# Autodesk Inventor assembly: Rail_AssemblyV2_0
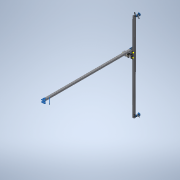
[picture p0: Inventor's stored thumbnail of the model, 180x180]
Saved by Autodesk Inventor 2021 (Build 250183000, 183)
## iProperties
Created: 2021-01-25
Part Number: Rail_AssemblyV2_0
Document SubType Name: Assembly
Designer: Jorian Brusind
Mass: 3786.54 g
Surface Area: 19508.5 cm^2
Volume: 2323.9 cm^3
Density: 1.62939 g/cm^3
Author: Jorian Brusind
## Documents named in this file (24)
- C:\Users\Jorian Brusind\Documents\GitHub\PersonalProjects\HyperRail\Inventor Files\Rail_AssemblyV2_0.iam
- C:\Users\Jorian Brusind\Documents\GitHub\PersonalProjects\Inventor Projects\Useful models\NEMA_Steppers\NEMA23\23HS8430B.ipt
- C:\Users\Jorian Brusind\Documents\GitHub\PersonalProjects\HyperRail\Inventor Files\NEMA23_StepperonlineMount.ipt
- C:\Users\Jorian Brusind\Documents\GitHub\PersonalProjects\Inventor Projects\Useful models\8020_Sets\IPT_20_Series\IPT_20_Series\20-2040_200mm.ipt
- C:\Users\Jorian Brusind\Documents\GitHub\PersonalProjects\HyperRail\Inventor Files\2804S_NEMA2115_1Gearbox.ipt
- C:\Users\Jorian Brusind\Documents\GitHub\PersonalProjects\Inventor Projects\Useful models\8020_Sets\IPT_40_Series\Extra_40_Series\90deg_4040.ipt
- C:\Users\Jorian Brusind\Documents\GitHub\PersonalProjects\HyperRail\Inventor Files\SmallBelt_LargePulley.ipt
- C:\Users\Jorian Brusind\Documents\GitHub\PersonalProjects\HyperRail\Inventor Files\Small_belt_5mm_1mm.ipt
- C:\Users\Jorian Brusind\Documents\GitHub\PersonalProjects\HyperRail\PCB Files\Integrated Stepper Motor Driver\ExportSTEP\Main.iam
- C:\Users\Jorian Brusind\Documents\GitHub\PersonalProjects\HyperRail\Inventor Files\NEMA23_Shroud.ipt
- C:\Users\Jorian Brusind\Documents\GitHub\PersonalProjects\Inventor Projects\Useful models\8020_Sets\IPT_20_Series\IPT_20_Series\20-4040_2m.ipt
- C:\Users\Jorian Brusind\Documents\GitHub\PersonalProjects\HyperRail\Inventor Files\98952A059_ALUM MALE-FEM THRDED HEX STANDOFF.ipt
- C:\Users\Jorian Brusind\Documents\GitHub\PersonalProjects\HyperRail\Inventor Files\95783A039_NYLON 6-6 MALE-FEM THRDED HEX STANDOFF.ipt
- C:\Users\Jorian Brusind\Documents\GitHub\PersonalProjects\HyperRail\Inventor Files\Integrated_Stepper_NEMA23_Mount.ipt
- C:\Users\Jorian Brusind\Documents\GitHub\PersonalProjects\HyperRail\Inventor Files\Foot_Spacer.ipt
- C:\Users\Jorian Brusind\Documents\GitHub\PersonalProjects\Inventor Projects\Useful models\Metric bolt\Bolt M5 50mm.ipt
- C:\Users\Jorian Brusind\Documents\GitHub\PersonalProjects\Inventor Projects\Useful models\Metric nuts\Nut M5.ipt
- C:\Users\Jorian Brusind\Documents\GitHub\PersonalProjects\HyperRail\Inventor Files\Bottom_Foot.ipt
- C:\Users\Jorian Brusind\Documents\GitHub\PersonalProjects\HyperRail\Inventor Files\120deg_Tslot_Gusset.ipt
- C:\Users\Jorian Brusind\Documents\GitHub\PersonalProjects\HyperRail\Inventor Files\90deg_4040Bracket.ipt
- C:\Users\Jorian Brusind\Documents\GitHub\PersonalProjects\HyperRail\Inventor Files\X_Carriage_V2_0.iam
- C:\Users\Jorian Brusind\Documents\GitHub\PersonalProjects\HyperRail\Inventor Files\11mm_BearingWheel.ipt
- C:\Users\Jorian Brusind\Documents\GitHub\PersonalProjects\HyperRail\Inventor Files\X_CarriageR_V2_0.iam
- C:\Users\Jorian Brusind\Documents\GitHub\PersonalProjects\HyperRail\Inventor Files\4mm_Roller_Spacer.ipt
## Components (40 placed, 23 different names)
1. 23HS8430B:1 — Mate:127, Angle:3, Mate:158, Mate:177, Mate:179, Mate:180, Mate:181, Mate:182, Mate:183, Mate:184, Mate:185, Mate:196, Mate:264, Mate:265
2. NEMA23_StepperonlineMount:1 — Angle:2, Mate:98, Mate:128, Mate:149, Mate:155, Flush:82, Mate:254, Mate:255, Mate:257, Mate:258, Mate:259, Mate:261, Mate:262
3. 20-2040_200mm:1 — Flush:34, Mate:83, Flush:35, Flush:36, Mate:85, Flush:56, Flush:63, Mate:151, Flush:82, Mate:252, Mate:253, Flush:83, Flush:84, Mate:256, Flush:85
4. 2804S_NEMA2115_1Gearbox:1 — Angle:2, Mate:98, Mate:109, Mate:127, Mate:128, Angle:3, Mate:158, Mate:204, Flush:66, Flush:86
5. 90deg_4040:1 — Flush:34, Mate:83, Flush:35, Mate:150
6. 90deg_4040:2 — Flush:36, Mate:85, Mate:149, Mate:152
7. SmallBelt_LargePulley:1 — Mate:204, Flush:66
8. Small_belt_5mm_1mm:1 — Mate:109, Flush:42, Mate:111, Flush:64
9. Small_belt_5mm_1mm:2 — Flush:42, Mate:111, Mate:154, Flush:64, Mate:205
10. Main:1 [sub-assembly] — Mate:199, Mate:267, Mate:268
11. 20-4040_2m:1 — Mate:139, Flush:56, Mate:154, Mate:205, Mate:243, Flush:76, Flush:77, Mate:248, Flush:79, Flush:80, Mate:252
12. 20-4040_2m:2 — Mate:150, Flush:63, Mate:151, Mate:152, Mate:155, Mate:230, Flush:69, Flush:70, Mate:231, Flush:71, Flush:72, Mate:232, Flush:73, Mate:233, Mate:234, Flush:74
13. NEMA23_Shroud:1 — Mate:264, Mate:265, Flush:86
14. 98952A059_ALUM MALE-FEM THRDED HEX STANDOFF:1 — Mate:180, Mate:181, Mate:186, Mate:191
15. 98952A059_ALUM MALE-FEM THRDED HEX STANDOFF:2 — Mate:184, Mate:185, Mate:189, Mate:192
16. 98952A059_ALUM MALE-FEM THRDED HEX STANDOFF:3 — Mate:177, Mate:179, Mate:187, Mate:190
17. 98952A059_ALUM MALE-FEM THRDED HEX STANDOFF:4 — Mate:182, Mate:183, Mate:188, Mate:193
18. 95783A039_NYLON 6-6 MALE-FEM THRDED HEX STANDOFF:1 — Mate:188, Mate:193, Angle:4
19. 95783A039_NYLON 6-6 MALE-FEM THRDED HEX STANDOFF:2 — Mate:186, Mate:191
20. 95783A039_NYLON 6-6 MALE-FEM THRDED HEX STANDOFF:3 — Mate:187, Mate:190, Mate:200
21. 95783A039_NYLON 6-6 MALE-FEM THRDED HEX STANDOFF:4 — Mate:189, Mate:192
22. Integrated_Stepper_NEMA23_Mount:1 — Mate:196, Mate:199, Mate:200, Angle:4, Mate:267, Mate:268
23. Bolt M5 50mm:1 — Mate:224, Mate:245, Mate:246, Mate:247, Mate:269
24. Nut M5:1 — Mate:226, Mate:247
25. Nut M5:2 — Mate:244, Flush:78, Mate:246
26. Bottom_Foot:1 — Mate:224, Mate:226, Mate:245, Flush:81
27. 120deg_Tslot_Gusset:1 — Mate:230, Flush:69, Flush:70
28. 120deg_Tslot_Gusset:2 — Mate:231, Flush:71, Flush:72
29. 90deg_4040Bracket:1 — Mate:232, Flush:73, Mate:233, Flush:75
30. 90deg_4040Bracket:2 — Mate:234, Flush:74, Flush:75
31. Foot_Spacer:1 — Mate:243, Flush:76, Flush:77, Mate:244, Flush:78, Mate:269
32. Foot_Spacer:2 — Mate:248, Flush:79, Flush:80, Mate:250
33. Bottom_Foot:2 — Mate:249, Mate:251, Flush:81
34. Bolt M5 50mm:2 — Mate:249, Mate:250, Mate:251
35. X_Carriage_V2_0:1 [sub-assembly] — Mate:253, Flush:83, Flush:84
36. 11mm_BearingWheel:1 — Mate:254, Mate:255, Mate:260
37. X_CarriageR_V2_0:1 [sub-assembly] — Mate:256, Flush:85, Mate:257
38. 11mm_BearingWheel:2 — Mate:258, Mate:259, Mate:263
39. 4mm_Roller_Spacer:1 — Mate:260, Mate:261
40. 4mm_Roller_Spacer:2 — Mate:262, Mate:263
## Relationships (98: Mate 69, Flush 26, Angle 3)
- Angle:2 (0 deg): NEMA23_StepperonlineMount:1 ↔ 2804S_NEMA2115_1Gearbox:1
- Flush:34: 20-2040_200mm:1 ↔ 90deg_4040:1
- Mate:83: 20-2040_200mm:1 ↔ 90deg_4040:1
- Flush:35: 20-2040_200mm:1 ↔ 90deg_4040:1
- Flush:36: 20-2040_200mm:1 ↔ 90deg_4040:2
- Mate:85: 20-2040_200mm:1 ↔ 90deg_4040:2
- Mate:98: NEMA23_StepperonlineMount:1 ↔ 2804S_NEMA2115_1Gearbox:1
- Mate:109 (10 mm): 2804S_NEMA2115_1Gearbox:1 ↔ Small_belt_5mm_1mm:1
- Flush:42: Small_belt_5mm_1mm:1 ↔ Small_belt_5mm_1mm:2
- Mate:111 (20 mm): Small_belt_5mm_1mm:1 ↔ Small_belt_5mm_1mm:2
- Mate:127: 23HS8430B:1 ↔ 2804S_NEMA2115_1Gearbox:1
- Mate:128: NEMA23_StepperonlineMount:1 ↔ 2804S_NEMA2115_1Gearbox:1
- Mate:139: 20-4040_2m:1
- Flush:56: 20-2040_200mm:1 ↔ 20-4040_2m:1
- Mate:149 (30 mm): NEMA23_StepperonlineMount:1 ↔ 90deg_4040:2
- Mate:150: 90deg_4040:1 ↔ 20-4040_2m:2
- Flush:63: 20-2040_200mm:1 ↔ 20-4040_2m:2
- Mate:151: 20-2040_200mm:1 ↔ 20-4040_2m:2
- Mate:152: 90deg_4040:2 ↔ 20-4040_2m:2
- Mate:154 (-10 mm): Small_belt_5mm_1mm:2 ↔ 20-4040_2m:1
- Flush:64: Small_belt_5mm_1mm:1 ↔ Small_belt_5mm_1mm:2
- Mate:155: NEMA23_StepperonlineMount:1 ↔ 20-4040_2m:2
- Angle:3 (0 deg): 23HS8430B:1 ↔ 2804S_NEMA2115_1Gearbox:1
- Mate:158: 23HS8430B:1 ↔ 2804S_NEMA2115_1Gearbox:1
- Mate:177: 23HS8430B:1 ↔ 98952A059_ALUM MALE-FEM THRDED HEX STANDOFF:3
- Mate:179: 23HS8430B:1 ↔ 98952A059_ALUM MALE-FEM THRDED HEX STANDOFF:3
- Mate:180: 23HS8430B:1 ↔ 98952A059_ALUM MALE-FEM THRDED HEX STANDOFF:1
- Mate:181: 23HS8430B:1 ↔ 98952A059_ALUM MALE-FEM THRDED HEX STANDOFF:1
- Mate:182: 23HS8430B:1 ↔ 98952A059_ALUM MALE-FEM THRDED HEX STANDOFF:4
- Mate:183: 23HS8430B:1 ↔ 98952A059_ALUM MALE-FEM THRDED HEX STANDOFF:4
- Mate:184: 23HS8430B:1 ↔ 98952A059_ALUM MALE-FEM THRDED HEX STANDOFF:2
- Mate:185: 23HS8430B:1 ↔ 98952A059_ALUM MALE-FEM THRDED HEX STANDOFF:2
- Mate:186: 98952A059_ALUM MALE-FEM THRDED HEX STANDOFF:1 ↔ 95783A039_NYLON 6-6 MALE-FEM THRDED HEX STANDOFF:2
- Mate:187: 98952A059_ALUM MALE-FEM THRDED HEX STANDOFF:3 ↔ 95783A039_NYLON 6-6 MALE-FEM THRDED HEX STANDOFF:3
- Mate:188: 98952A059_ALUM MALE-FEM THRDED HEX STANDOFF:4 ↔ 95783A039_NYLON 6-6 MALE-FEM THRDED HEX STANDOFF:1
- Mate:189: 98952A059_ALUM MALE-FEM THRDED HEX STANDOFF:2 ↔ 95783A039_NYLON 6-6 MALE-FEM THRDED HEX STANDOFF:4
- Mate:190: 98952A059_ALUM MALE-FEM THRDED HEX STANDOFF:3 ↔ 95783A039_NYLON 6-6 MALE-FEM THRDED HEX STANDOFF:3
- Mate:191: 98952A059_ALUM MALE-FEM THRDED HEX STANDOFF:1 ↔ 95783A039_NYLON 6-6 MALE-FEM THRDED HEX STANDOFF:2
- Mate:192: 98952A059_ALUM MALE-FEM THRDED HEX STANDOFF:2 ↔ 95783A039_NYLON 6-6 MALE-FEM THRDED HEX STANDOFF:4
- Mate:193: 98952A059_ALUM MALE-FEM THRDED HEX STANDOFF:4 ↔ 95783A039_NYLON 6-6 MALE-FEM THRDED HEX STANDOFF:1
- Mate:196 (2 mm): 23HS8430B:1 ↔ Integrated_Stepper_NEMA23_Mount:1
- Mate:199 (1 mm): Main:1 ↔ Integrated_Stepper_NEMA23_Mount:1
- Mate:200: 95783A039_NYLON 6-6 MALE-FEM THRDED HEX STANDOFF:3 ↔ Integrated_Stepper_NEMA23_Mount:1
- Angle:4 (0 deg): 95783A039_NYLON 6-6 MALE-FEM THRDED HEX STANDOFF:1 ↔ Integrated_Stepper_NEMA23_Mount:1
- Mate:204: 2804S_NEMA2115_1Gearbox:1 ↔ SmallBelt_LargePulley:1
- Flush:66: 2804S_NEMA2115_1Gearbox:1 ↔ SmallBelt_LargePulley:1
- Mate:205: Small_belt_5mm_1mm:2 ↔ 20-4040_2m:1
- Mate:224: Bolt M5 50mm:1 ↔ Bottom_Foot:1
- Mate:226: Nut M5:1 ↔ Bottom_Foot:1
- Mate:230: 20-4040_2m:2 ↔ 120deg_Tslot_Gusset:1
- Flush:69: 20-4040_2m:2 ↔ 120deg_Tslot_Gusset:1
- Flush:70: 20-4040_2m:2 ↔ 120deg_Tslot_Gusset:1
- Mate:231: 20-4040_2m:2 ↔ 120deg_Tslot_Gusset:2
- Flush:71: 20-4040_2m:2 ↔ 120deg_Tslot_Gusset:2
- Flush:72: 20-4040_2m:2 ↔ 120deg_Tslot_Gusset:2
- Mate:232: 20-4040_2m:2 ↔ 90deg_4040Bracket:1
- Flush:73: 20-4040_2m:2 ↔ 90deg_4040Bracket:1
- Mate:233: 20-4040_2m:2 ↔ 90deg_4040Bracket:1
- Mate:234: 20-4040_2m:2 ↔ 90deg_4040Bracket:2
- Flush:74: 20-4040_2m:2 ↔ 90deg_4040Bracket:2
- Flush:75: 90deg_4040Bracket:1 ↔ 90deg_4040Bracket:2
- Mate:243: 20-4040_2m:1 ↔ Foot_Spacer:1
- Flush:76: 20-4040_2m:1 ↔ Foot_Spacer:1
- Flush:77: 20-4040_2m:1 ↔ Foot_Spacer:1
- Mate:244: Nut M5:2 ↔ Foot_Spacer:1
- Flush:78: Nut M5:2 ↔ Foot_Spacer:1
- Mate:245: Bolt M5 50mm:1 ↔ Bottom_Foot:1
- Mate:246: Bolt M5 50mm:1 ↔ Nut M5:2
- Mate:247: Bolt M5 50mm:1 ↔ Nut M5:1
- Mate:248: 20-4040_2m:1 ↔ Foot_Spacer:2
- Flush:79: 20-4040_2m:1 ↔ Foot_Spacer:2
- Flush:80: 20-4040_2m:1 ↔ Foot_Spacer:2
- Mate:249: Bottom_Foot:2 ↔ Bolt M5 50mm:2
- Mate:250: Foot_Spacer:2 ↔ Bolt M5 50mm:2
- Mate:251: Bottom_Foot:2 ↔ Bolt M5 50mm:2
- Flush:81: Bottom_Foot:1 ↔ Bottom_Foot:2
- Flush:82 (1 mm): NEMA23_StepperonlineMount:1 ↔ 20-2040_200mm:1
- Mate:252 (8 mm): 20-2040_200mm:1 ↔ 20-4040_2m:1
- Mate:253: 20-2040_200mm:1 ↔ X_Carriage_V2_0:1
- Flush:83 (-23 mm): 20-2040_200mm:1 ↔ X_Carriage_V2_0:1
- Flush:84: 20-2040_200mm:1 ↔ X_Carriage_V2_0:1
- Mate:254: NEMA23_StepperonlineMount:1 ↔ 11mm_BearingWheel:1
- Mate:255 (13 mm): NEMA23_StepperonlineMount:1 ↔ 11mm_BearingWheel:1
- Mate:256: 20-2040_200mm:1 ↔ X_CarriageR_V2_0:1
- Flush:85 (-23 mm): 20-2040_200mm:1 ↔ X_CarriageR_V2_0:1
- Mate:257 (-18.5 mm): NEMA23_StepperonlineMount:1 ↔ X_CarriageR_V2_0:1
- Mate:258: NEMA23_StepperonlineMount:1 ↔ 11mm_BearingWheel:2
- Mate:259 (13 mm): NEMA23_StepperonlineMount:1 ↔ 11mm_BearingWheel:2
- Mate:260: 11mm_BearingWheel:1 ↔ 4mm_Roller_Spacer:1
- Mate:261: NEMA23_StepperonlineMount:1 ↔ 4mm_Roller_Spacer:1
- Mate:262: NEMA23_StepperonlineMount:1 ↔ 4mm_Roller_Spacer:2
- Mate:263: 11mm_BearingWheel:2 ↔ 4mm_Roller_Spacer:2
- Mate:264 (1 mm): 23HS8430B:1 ↔ NEMA23_Shroud:1
- Mate:265 (1 mm): 23HS8430B:1 ↔ NEMA23_Shroud:1
- Mate:267: Main:1 ↔ Integrated_Stepper_NEMA23_Mount:1
- Mate:268: Main:1 ↔ Integrated_Stepper_NEMA23_Mount:1
- Mate:269: Bolt M5 50mm:1 ↔ Foot_Spacer:1
- Flush:86: 2804S_NEMA2115_1Gearbox:1 ↔ NEMA23_Shroud:1
